# Autodesk Inventor assembly: LearnbotDefinitivo
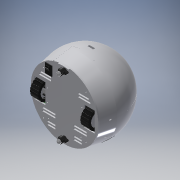
[picture p0: Inventor's stored thumbnail of the model, 180x180]
Saved by Autodesk Inventor 2017 (Build 210142000, 142)
## iProperties
Part Number: LearnbotDefinitivo
Material: Genérico
Document SubType Name: Assembly
Designer: Roberto
Author: Roberto
## Documents named in this file (22)
- C:\Users\Roberto\Desktop\learnbotPruebas\LearnbotAssembly.iam
- C:\Users\Roberto\Desktop\learnbotPruebas\LearnbotBase.ipt
- C:\Users\Roberto\Desktop\learnbotPruebas\LearnbotBatteryBase.ipt
- C:\Users\Roberto\Desktop\learnbotPruebas\learnbotSupportMotor.ipt
- C:\Users\Roberto\Desktop\learnbotPruebas\learnbotWheel.ipt
- C:\Users\Roberto\Desktop\learnbotPruebas\LearnbotBattery.ipt
- C:\Users\Roberto\Desktop\learnbotPruebas\LearnbotSupportOdroid.ipt
- C:\Users\Roberto\Desktop\learnbotPruebas\learnbotOdroid.ipt
- C:\Users\Roberto\Desktop\learnbotPruebas\LearnbotSupportScreen##.ipt
- C:\Users\Roberto\Desktop\learnbotPruebas\LearnbotScreen.ipt
- C:\Users\Roberto\Desktop\learnbotPruebas\learnbotCasterBall.ipt
- C:\Users\Roberto\Desktop\learnbotPruebas\LearnbotSwitch.ipt
- C:\Users\Roberto\Desktop\learnbotPruebas\LearnbotSupportCameraA.ipt
- C:\Users\Roberto\Desktop\learnbotPruebas\learnbotServo.ipt
- C:\Users\Roberto\Desktop\learnbotPruebas\learnbotPieceServo.ipt
- C:\Users\Roberto\Desktop\learnbotPruebas\LearnbotSupportCameraB.ipt
- C:\Users\Roberto\Desktop\learnbotPruebas\LearnbotCamera.ipt
- C:\Users\Roberto\Desktop\learnbotPruebas\LearnbotBack.ipt
- C:\Users\Roberto\Desktop\learnbotPruebas\LearnbotFront.ipt
- C:\Users\Roberto\Desktop\learnbotPruebas\LearnbotLaser.ipt
- C:\Users\Roberto\Desktop\learnbotPruebas\LearnbotBackCoverScreen#.ipt
- C:\Users\Roberto\Desktop\learnbotPruebas\LearnbotCristal###.ipt
## Components (31 placed, 21 different names)
1. LearnbotBase:1 — Coincidencia:1, Coincidencia:2, Coincidencia:3, Coincidencia:4, Coincidencia:5, Coincidencia:11, Coincidencia:19, Coincidencia:23, Coincidencia:26, Coincidencia:27, Coincidencia:32, Coincidencia:66
2. LearnbotBatteryBase:1 — Coincidencia:3, Coincidencia:4, Coincidencia:5, Coincidencia:8, Coincidencia:9, Coincidencia:24
3. learnbotSupportMotor:1 — Coincidencia:1, Coincidencia:7, Coincidencia:10, Coincidencia:11
4. learnbotSupportMotor:2 — Coincidencia:2, Coincidencia:6, Coincidencia:12
5. learnbotWheel:1 — Coincidencia:6
6. learnbotWheel:2 — Coincidencia:7
7. LearnbotBattery:1 — Coincidencia:8, Coincidencia:9
8. LearnbotSupportOdroid:1 — Coincidencia:12
9. LearnbotSupportOdroid:2 — Coincidencia:10, Coincidencia:42
10. learnbotOdroid:1 — Coincidencia:42
11. LearnbotSupportScreen##:1 — Coincidencia:19, Coincidencia:32, Coincidencia:43, Coincidencia:44, Coincidencia:45, Coincidencia:46, Coincidencia:47
12. learnbotCasterBall:1 — Coincidencia:23
13. learnbotCasterBall:2 — Coincidencia:24
14. LearnbotSwitch:1 — Coincidencia:26, Coincidencia:27
15. LearnbotSupportCameraA:1 — Coincidencia:35, Coincidencia:37
16. learnbotServo:1 — Coincidencia:35, Coincidencia:36, Coincidencia:37, Coincidencia:38
17. learnbotPieceServo:1 — Coincidencia:36, Coincidencia:38, Coincidencia:39, Coincidencia:40
18. LearnbotSupportCameraB:1 — Coincidencia:39, Coincidencia:40, Coincidencia:41
19. LearnbotCamera:1 — Coincidencia:41
20. LearnbotScreen:1 — Coincidencia:43, Coincidencia:44, Coincidencia:45, Coincidencia:46, Coincidencia:47, Coincidencia:64, Coincidencia:65
21. LearnbotFront:1 — Coincidencia:48, Coincidencia:49, Coincidencia:50, Coincidencia:51, Coincidencia:52, Coincidencia:53, Coincidencia:54, Coincidencia:55, Coincidencia:56, Coincidencia:57, Coincidencia:58, Coincidencia:59, Coincidencia:60, Coincidencia:67, Coincidencia:68, Coincidencia:69
22. LearnbotLaser:1 — Coincidencia:51
23. LearnbotLaser:2 — Coincidencia:50
24. LearnbotLaser:4 — Coincidencia:54, Coincidencia:55
25. LearnbotLaser:5 — Coincidencia:52, Coincidencia:53
26. LearnbotLaser:6 — Coincidencia:48, Coincidencia:49
27. LearnbotLaser:7 — Coincidencia:59, Coincidencia:60
28. LearnbotLaser:8 — Coincidencia:56, Coincidencia:57, Coincidencia:58
29. LearnbotBackCoverScreen#:1 — Coincidencia:64, Coincidencia:65
30. LearnbotBack:1 — Coincidencia:66
31. LearnbotCristal###:1 — Coincidencia:67, Coincidencia:68, Coincidencia:69
## Relationships (50: Mate 50)
- Coincidencia:1 [Mate]: LearnbotBase:1 ↔ learnbotSupportMotor:1
- Coincidencia:2 [Mate]: LearnbotBase:1 ↔ learnbotSupportMotor:2
- Coincidencia:3 [Mate]: LearnbotBase:1 ↔ LearnbotBatteryBase:1
- Coincidencia:4 [Mate]: LearnbotBase:1 ↔ LearnbotBatteryBase:1
- Coincidencia:5 [Mate]: LearnbotBase:1 ↔ LearnbotBatteryBase:1
- Coincidencia:6 [Mate]: learnbotSupportMotor:2 ↔ learnbotWheel:1
- Coincidencia:7 [Mate]: learnbotSupportMotor:1 ↔ learnbotWheel:2
- Coincidencia:8 [Mate]: LearnbotBatteryBase:1 ↔ LearnbotBattery:1
- Coincidencia:9 [Mate]: LearnbotBatteryBase:1 ↔ LearnbotBattery:1
- Coincidencia:10 [Mate]: learnbotSupportMotor:1 ↔ LearnbotSupportOdroid:2
- Coincidencia:11 [Mate]: LearnbotBase:1 ↔ learnbotSupportMotor:1
- Coincidencia:12 [Mate]: learnbotSupportMotor:2 ↔ LearnbotSupportOdroid:1
- Coincidencia:19 [Mate]: LearnbotBase:1 ↔ LearnbotSupportScreen##:1
- Coincidencia:23 [Mate]: LearnbotBase:1 ↔ learnbotCasterBall:1
- Coincidencia:24 [Mate]: LearnbotBatteryBase:1 ↔ learnbotCasterBall:2
- Coincidencia:26 [Mate]: LearnbotBase:1 ↔ LearnbotSwitch:1
- Coincidencia:27 [Mate]: LearnbotBase:1 ↔ LearnbotSwitch:1
- Coincidencia:32 [Mate]: LearnbotBase:1 ↔ LearnbotSupportScreen##:1
- Coincidencia:35 [Mate]: LearnbotSupportCameraA:1 ↔ learnbotServo:1
- Coincidencia:36 [Mate]: learnbotServo:1 ↔ learnbotPieceServo:1
- Coincidencia:37 [Mate]: LearnbotSupportCameraA:1 ↔ learnbotServo:1
- Coincidencia:38 [Mate]: learnbotServo:1 ↔ learnbotPieceServo:1
- Coincidencia:39 [Mate]: learnbotPieceServo:1 ↔ LearnbotSupportCameraB:1
- Coincidencia:40 [Mate]: learnbotPieceServo:1 ↔ LearnbotSupportCameraB:1
- Coincidencia:41 [Mate]: LearnbotSupportCameraB:1 ↔ LearnbotCamera:1
- Coincidencia:42 [Mate]: LearnbotSupportOdroid:2 ↔ learnbotOdroid:1
- Coincidencia:43 [Mate]: LearnbotSupportScreen##:1 ↔ LearnbotScreen:1
- Coincidencia:44 [Mate]: LearnbotSupportScreen##:1 ↔ LearnbotScreen:1
- Coincidencia:45 [Mate]: LearnbotSupportScreen##:1 ↔ LearnbotScreen:1
- Coincidencia:46 [Mate]: LearnbotSupportScreen##:1 ↔ LearnbotScreen:1
- Coincidencia:47 [Mate]: LearnbotSupportScreen##:1 ↔ LearnbotScreen:1
- Coincidencia:48 [Mate]: LearnbotFront:1 ↔ LearnbotLaser:6
- Coincidencia:49 [Mate]: LearnbotFront:1 ↔ LearnbotLaser:6
- Coincidencia:50 [Mate]: LearnbotFront:1 ↔ LearnbotLaser:2
- Coincidencia:51 [Mate]: LearnbotFront:1 ↔ LearnbotLaser:1
- Coincidencia:52 [Mate]: LearnbotFront:1 ↔ LearnbotLaser:5
- Coincidencia:53 [Mate]: LearnbotFront:1 ↔ LearnbotLaser:5
- Coincidencia:54 [Mate]: LearnbotFront:1 ↔ LearnbotLaser:4
- Coincidencia:55 [Mate]: LearnbotFront:1 ↔ LearnbotLaser:4
- Coincidencia:56 [Mate]: LearnbotFront:1 ↔ LearnbotLaser:8
- Coincidencia:57 [Mate]: LearnbotFront:1 ↔ LearnbotLaser:8
- Coincidencia:58 [Mate]: LearnbotFront:1 ↔ LearnbotLaser:8
- Coincidencia:59 [Mate]: LearnbotFront:1 ↔ LearnbotLaser:7
- Coincidencia:60 [Mate]: LearnbotFront:1 ↔ LearnbotLaser:7
- Coincidencia:64 [Mate]: LearnbotScreen:1 ↔ LearnbotBackCoverScreen#:1
- Coincidencia:65 [Mate]: LearnbotScreen:1 ↔ LearnbotBackCoverScreen#:1
- Coincidencia:66 [Mate]: LearnbotBase:1 ↔ LearnbotBack:1
- Coincidencia:67 [Mate]: LearnbotFront:1 ↔ LearnbotCristal###:1
- Coincidencia:68 [Mate]: LearnbotFront:1 ↔ LearnbotCristal###:1
- Coincidencia:69 [Mate]: LearnbotFront:1 ↔ LearnbotCristal###:1
